# Autodesk Inventor assembly: GameBoy
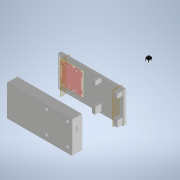
[picture p0: Inventor's stored thumbnail of the model, 180x180]
Saved by Autodesk Inventor 2022 (Build 260153000, 153)
## iProperties
Created: 2023-09-02
Part Number: GameBoy
Document SubType Name: Assembly
Designer: Petr Černý
Author: Petr Černý
## Documents named in this file (8)
- C:\Projekty\GameBoy\Enclosure_3D\3D Model\GameBoy.iam
- C:\Projekty\GameBoy\Enclosure_3D\3D Model\LowerHalf.ipt
- C:\Projekty\GameBoy\Enclosure_3D\3D Model\Upper_Half.ipt
- C:\Projekty\GameBoy\Enclosure_3D\3D Model\GameBoy_PCB.iam
- C:\Projekty\GameBoy\Enclosure_3D\3D Model\Nokia5110.iam
- C:\Projekty\GameBoy\Enclosure_3D\3D Model\Tactile_Push_Button.ipt
- C:\Projekty\GameBoy\Enclosure_3D\3D Model\BatteryDoor.ipt
- C:\Projekty\GameBoy\Enclosure_3D\3D Model\9V-battery.ipt
## Components (7 placed, 7 different names)
1. LowerHalf:1 — Mate:33, Mate:34, Mate:35, Mate:37, Mate:38, Mate:39, Mate:40, Mate:41
2. Upper_Half:1
3. Nokia5110:1 [sub-assembly]
4. BatteryDoor:1 — Mate:33, Mate:34, Mate:35, Mate:36
5. GameBoy_PCB:1 [sub-assembly] — Mate:39, Mate:40, Mate:41
6. 9V-battery:1 — Mate:36, Mate:37, Mate:38
7. Tactile_Push_Button:1
## Relationships (10: Mate 9, Flush 1)
- Mate:33: LowerHalf:1 ↔ BatteryDoor:1
- Mate:34: LowerHalf:1 ↔ BatteryDoor:1
- Mate:35: LowerHalf:1 ↔ BatteryDoor:1
- Mate:36: BatteryDoor:1 ↔ 9V-battery:1
- Mate:37 (10 mm): LowerHalf:1 ↔ 9V-battery:1
- Mate:38 (15 mm): LowerHalf:1 ↔ 9V-battery:1
- Mate:39: LowerHalf:1 ↔ GameBoy_PCB:1
- Mate:40 (1.5 mm): LowerHalf:1 ↔ GameBoy_PCB:1
- Mate:41 (1 mm): LowerHalf:1 ↔ GameBoy_PCB:1
- Flush:12 (-100 mm)
